# Autodesk Inventor assembly: BottomPlate
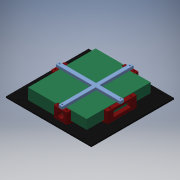
[picture p0: Inventor's stored thumbnail of the model, 180x180]
Saved by Autodesk Inventor 2016 (Build 200138000, 138)
## iProperties
Created: 2015-09-23
Part Number: BottomPlate
Document SubType Name: Assembly
Designer: lachesis
Author: lachesis
## Documents named in this file (3)
- C:\Users\lachesis\git\Swarmie-Build\Swarmie-Assembly\Assemblies\BottomPlate.iam
- C:\Users\lachesis\git\Swarmie-Build\Swarmie-Assembly\Parts\BottomPlate - Copy.ipt
- C:\Users\lachesis\git\Swarmie-Build\Swarmie-Assembly\Assemblies\Battery.iam
## Components (2 placed, 2 different names)
1. BottomPlate - Copy:1 — Rigid:1
2. Battery:1 [sub-assembly] — Rigid:1
## Relationships (1: WeldJoint 1)
- Rigid:1 [WeldJoint]: BottomPlate - Copy:1 ↔ Battery:1
